# Autodesk Inventor assembly: 脚ギア1段目
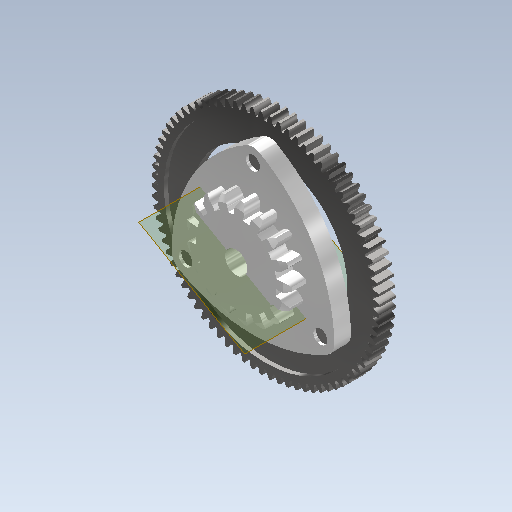
[picture p0: Inventor's stored thumbnail of the model, 512x512]
Saved by Autodesk Inventor 2020.4 (Build 244396000, 396)
## iProperties
Created: 2020-10-28
Part Number: 脚ギア1段目
Document SubType Name: Assembly
Designer: AA19065
Mass: 18.8119 g
Surface Area: 48.6042 cm^2
Volume: 3.94374 cm^3
Density: 4.77006 g/cm^3
Author: AA19065
## Documents named in this file (4)
- C:\Users\happy\OneDrive\ドキュメント\賢一ファイル\SRDC\試作10-2\アセンブリ\脚ギア1段目.iam
- C:\Users\happy\OneDrive\ドキュメント\賢一ファイル\SRDC\試作10-2\ギア\m1z17.ipt
- C:\Users\happy\OneDrive\ドキュメント\賢一ファイル\SRDC\試作10-2\ギア\歯車m0.5,z80.ipt
- C:\Users\happy\OneDrive\ドキュメント\賢一ファイル\SRDC\試作10-2\ねじ\M3L4　超極低頭.ipt
## Components (5 placed, 3 different names)
1. m1z17:1 — 挿入:1, 挿入:2
2. 歯車m0.5,z80:1 — 挿入:1, 挿入:2, 挿入:3, 挿入:4, 挿入:5
3. M3L4　超極低頭:1 — 挿入:3
4. M3L4　超極低頭:2 — 挿入:4
5. M3L4　超極低頭:3 — 挿入:5
## Relationships (5: Insert 5)
- 挿入:1 [Insert]: m1z17:1 ↔ 歯車m0.5,z80:1
- 挿入:2 [Insert]: m1z17:1 ↔ 歯車m0.5,z80:1
- 挿入:3 [Insert]: 歯車m0.5,z80:1 ↔ M3L4　超極低頭:1
- 挿入:4 [Insert]: 歯車m0.5,z80:1 ↔ M3L4　超極低頭:2
- 挿入:5 [Insert]: 歯車m0.5,z80:1 ↔ M3L4　超極低頭:3
